# Autodesk Inventor assembly: DD_KVD_009
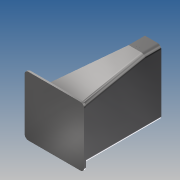
[picture p0: Inventor's stored thumbnail of the model, 180x180]
Saved by Autodesk Inventor 2017.3 (Build 213256000, 256)
## iProperties
Created: 2023-12-08
Part Number: DD_KVD_009
Document SubType Name: Weldment
Designer: Darena
Weld Material: Nerezová ocel
Author: Darena
## Documents named in this file (3)
- D:\2_Darena\1_Soukrome\02_Inventor soukromé\Dílna RAKO3\Záhora\Pivovar KONTEJNER\S výklopným dnem\DD_KVD_001\DD_KVD_009.iam
- D:\2_Darena\1_Soukrome\02_Inventor soukromé\Dílna RAKO3\Záhora\Pivovar KONTEJNER\S výklopným dnem\DD_KVD_001\DD_KVD_003_09_A.ipt
- D:\2_Darena\1_Soukrome\02_Inventor soukromé\Dílna RAKO3\Záhora\Pivovar KONTEJNER\S výklopným dnem\DD_KVD_001\DD_KVD_003_09_B.ipt
## Components (2 placed, 2 different names)
1. DD_KVD_003_09_A:1 — Proti sobě:3, Stejný směr:2, Proti sobě:4
2. DD_KVD_003_09_B:1 — Proti sobě:1, Proti sobě:2, Stejný směr:1, Proti sobě:3
## Relationships (6: Mate 4, Flush 2)
- Proti sobě:1 [Mate]: DD_KVD_003_09_B:1
- Proti sobě:2 [Mate]: DD_KVD_003_09_B:1
- Stejný směr:1 [Flush]: DD_KVD_003_09_B:1
- Proti sobě:3 [Mate]: DD_KVD_003_09_A:1 ↔ DD_KVD_003_09_B:1
- Stejný směr:2 [Flush] (-5 mm): DD_KVD_003_09_A:1
- Proti sobě:4 [Mate] (5 mm): DD_KVD_003_09_A:1
